# Autodesk Inventor assembly: Collector rotator assembly for extension arm
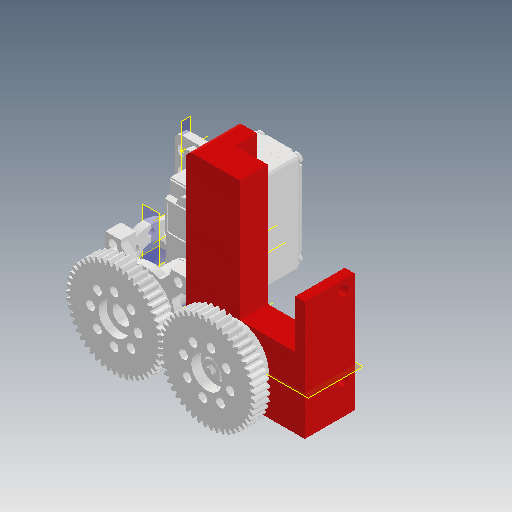
[picture p0: Inventor's stored thumbnail of the model, 512x512]
Saved by Autodesk Inventor 2020 (Build 240168000, 168)
## iProperties
Created: 2020-01-01
Part Number: Collector rotator assembly for extension arm
Document SubType Name: Assembly
Designer: ball
Author: ball
## Documents named in this file (5)
- C:\FTC\FTC8863CAD\2019 Robot\Collection\Collector rotator assembly for extension arm.iam
- C:\FTC\FTC8863CAD\2019 Robot\Collection\Collector mount adapter.ipt
- C:\FTC\FTC8863CAD\2019 Robot\Collection\turntable + gear.iam
- C:\FTC\FTC8863CAD\2019 Robot\Collection\Servo block + gear.iam
- C:\FTC\FTC8863CAD\StepLibraries\Screws\6-32x.375_18-8 SS TRUSS HEAD PHILLIPS MACHINE SCREW.ipt
## Components (5 placed, 4 different names)
1. Collector mount adapter:1 — Mate:1, Mate:2, Flush:2, Mate:3, Mate:4, Mate:7, Mate:8, Mate:9, Mate:10
2. turntable + gear:1 [sub-assembly] — Mate:1, Flush:1, Mate:3, Mate:4
3. Servo block + gear:1 [sub-assembly] — Flush:1, Mate:2, Flush:2
4. 6-32x.375_18-8 SS TRUSS HEAD PHILLIPS MACHINE SCREW:1 — Mate:7, Mate:8
5. 6-32x.375_18-8 SS TRUSS HEAD PHILLIPS MACHINE SCREW:2 — Mate:9, Mate:10
## Relationships (10: Mate 8, Flush 2)
- Mate:1: Collector mount adapter:1 ↔ turntable + gear:1
- Flush:1: turntable + gear:1 ↔ Servo block + gear:1
- Mate:2: Collector mount adapter:1 ↔ Servo block + gear:1
- Flush:2: Collector mount adapter:1 ↔ Servo block + gear:1
- Mate:3: Collector mount adapter:1 ↔ turntable + gear:1
- Mate:4: Collector mount adapter:1 ↔ turntable + gear:1
- Mate:7: Collector mount adapter:1 ↔ 6-32x.375_18-8 SS TRUSS HEAD PHILLIPS MACHINE SCREW:1
- Mate:8: Collector mount adapter:1 ↔ 6-32x.375_18-8 SS TRUSS HEAD PHILLIPS MACHINE SCREW:1
- Mate:9: Collector mount adapter:1 ↔ 6-32x.375_18-8 SS TRUSS HEAD PHILLIPS MACHINE SCREW:2
- Mate:10: Collector mount adapter:1 ↔ 6-32x.375_18-8 SS TRUSS HEAD PHILLIPS MACHINE SCREW:2
